# Autodesk Inventor assembly: Plataforma 4dof
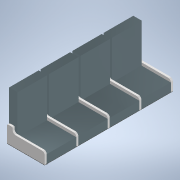
[picture p0: Inventor's stored thumbnail of the model, 180x180]
Saved by Autodesk Inventor 2021 (Build 250183000, 183)
## iProperties
Created: 2021-03-18
Part Number: Plataforma 4dof
Document SubType Name: Assembly
Designer: andre
Author: andre
## Documents named in this file (5)
- C:\Users\andre\Documents\GitHub\Dis.-Mecatronico-E6\Inventor\Plataforma 4dof.iam
- C:\Users\andre\Documents\GitHub\Dis.-Mecatronico-E6\Inventor\placa inferior.ipt
- C:\Users\andre\Documents\GitHub\Dis.-Mecatronico-E6\Inventor\placa superior.ipt
- C:\Users\andre\Documents\GitHub\Dis.-Mecatronico-E6\Inventor\silla.ipt
- C:\Users\andre\Documents\GitHub\Dis.-Mecatronico-E6\Inventor\bracera.ipt
## Components (11 placed, 4 different names)
1. placa inferior:1 — Flush:1
2. placa superior:1 — Flush:2, Flush:3, Flush:4, Flush:5, Mate:1, Mate:2, Mate:3, Mate:4
3. silla:1 — Flush:4, Flush:5, Mate:1, Rigid:1, Rigid:2
4. silla:2 — Mate:2, Rigid:3, Rigid:4
5. silla:3 — Mate:3, Rigid:5, Rigid:6
6. silla:4 — Mate:4, Rigid:7, Rigid:8
7. bracera:1 — Rigid:1
8. bracera:2 — Rigid:2, Rigid:3
9. bracera:3 — Rigid:4, Rigid:5
10. bracera:4 — Rigid:6, Rigid:7
11. bracera:5 — Rigid:8
## Relationships (17: WeldJoint 8, Flush 5, Mate 4)
- Flush:1 (600 mm): placa inferior:1
- Flush:2: placa superior:1
- Flush:3: placa superior:1
- Flush:4: placa superior:1 ↔ silla:1
- Flush:5: placa superior:1 ↔ silla:1
- Mate:1: placa superior:1 ↔ silla:1
- Mate:2: placa superior:1 ↔ silla:2
- Mate:3: placa superior:1 ↔ silla:3
- Mate:4: placa superior:1 ↔ silla:4
- Rigid:1 [WeldJoint]: silla:1 ↔ bracera:1
- Rigid:2 [WeldJoint]: silla:1 ↔ bracera:2
- Rigid:3 [WeldJoint]: silla:2 ↔ bracera:2
- Rigid:4 [WeldJoint]: silla:2 ↔ bracera:3
- Rigid:5 [WeldJoint]: silla:3 ↔ bracera:3
- Rigid:6 [WeldJoint]: silla:3 ↔ bracera:4
- Rigid:7 [WeldJoint]: silla:4 ↔ bracera:4
- Rigid:8 [WeldJoint]: silla:4 ↔ bracera:5
